# Autodesk Inventor assembly: Toughbox-mini box
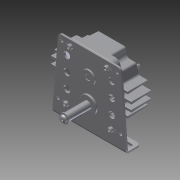
[picture p0: Inventor's stored thumbnail of the model, 180x180]
Saved by Autodesk Inventor 2014 SP1 (Build 180222100, 222)
## iProperties
Created: 2014-01-21
Part Number: Toughbox-mini box
Document SubType Name: Assembly
Designer: Nick
Translation Standard: STEP AP203
FileName: S:/Products/Gearboxes Spur Single Stage/Toughbox/Toughbox Mini/Toughbox-Mini.stp
PreProcessor: Unknown
PostProcessor: Build: 160, Release: 2012 RTM - Date: Tue 03/01/2011
Sent Units: millimeter
Uncertainty: 0.001
Author: Nick
## Documents named in this file (20)
- D:\Dropbox\School\PurdueFIRST\PFP Robot\PFP Robot with Cart\Toughbox-mini box.iam
- D:\Dropbox\School\PurdueFIRST\PFP Robot\PFP Robot with Cart\r6zz.ipt
- D:\Dropbox\School\PurdueFIRST\PFP Robot\PFP Robot with Cart\Toughbox_d03.ipt
- D:\Dropbox\School\PurdueFIRST\PFP Robot\PFP Robot with Cart\Toughbox_d07.ipt
- D:\Dropbox\School\PurdueFIRST\PFP Robot\PFP Robot with Cart\Toughbox_d05.ipt
- D:\Dropbox\School\PurdueFIRST\PFP Robot\PFP Robot with Cart\Toughbox_d08.ipt
- D:\Dropbox\School\PurdueFIRST\PFP Robot\PFP Robot with Cart\Toughbox_d06.ipt
- D:\Dropbox\School\PurdueFIRST\PFP Robot\PFP Robot with Cart\fr-6-zz.ipt
- D:\Dropbox\School\PurdueFIRST\PFP Robot\PFP Robot with Cart\fr-8-zz.ipt
- D:\Dropbox\School\PurdueFIRST\PFP Robot\PFP Robot with Cart\10-32_nylock_nut.ipt
- D:\Dropbox\School\PurdueFIRST\PFP Robot\PFP Robot with Cart\5-16_washer.ipt
- D:\Dropbox\School\PurdueFIRST\PFP Robot\PFP Robot with Cart\Toughbox_d09.ipt
- D:\Dropbox\School\PurdueFIRST\PFP Robot\PFP Robot with Cart\8mm_spring_clip.ipt
- D:\Dropbox\School\PurdueFIRST\PFP Robot\PFP Robot with Cart\Toughbox-mini_d01-5-12.ipt
- D:\Dropbox\School\PurdueFIRST\PFP Robot\PFP Robot with Cart\Toughbox-mini_d02.ipt
- D:\Dropbox\School\PurdueFIRST\PFP Robot\PFP Robot with Cart\250_washer.ipt
- D:\Dropbox\School\PurdueFIRST\PFP Robot\PFP Robot with Cart\14-20x0500_bhcs.ipt
- D:\Dropbox\School\PurdueFIRST\PFP Robot\PFP Robot with Cart\125x124x700_key.ipt
- D:\Dropbox\School\PurdueFIRST\PFP Robot\PFP Robot with Cart\10-32x0625_shcs.ipt
- D:\Dropbox\School\PurdueFIRST\PFP Robot\PFP Robot with Cart\TB Output Shaft AM14U.ipt
## Components (35 placed, 19 different names)
1. r6zz:1
2. r6zz:2
3. Toughbox_d03:1
4. Toughbox_d07:1
5. Toughbox_d05:1
6. Toughbox_d08:1
7. Toughbox_d06:1
8. fr-6-zz:1
9. fr-8-zz:1
10. 10-32_nylock_nut:1
11. 10-32_nylock_nut:2
12. 10-32_nylock_nut:3
13. 10-32_nylock_nut:4
14. 5-16_washer:1
15. 5-16_washer:2
16. 5-16_washer:3
17. 5-16_washer:4
18. Toughbox_d09:1
19. Toughbox_d09:2
20. 8mm_spring_clip:1
21. 8mm_spring_clip:2
22. Toughbox-mini_d01-5-12:1 — Insert:1
23. Toughbox-mini_d02:1
24. 250_washer:1
25. 14-20x0500_bhcs:1
26. 125x124x700_key:1
27. 10-32x0625_shcs:1
28. 10-32x0625_shcs:2
29. 10-32x0625_shcs:3
30. 10-32x0625_shcs:4
31. 10-32x0625_shcs:5
32. 10-32x0625_shcs:6
33. 10-32x0625_shcs:7
34. 10-32x0625_shcs:8
35. TB Output Shaft AM14U:1 — Insert:1
## Relationships (1: Insert 1)
- Insert:1 (-8.636 mm): Toughbox-mini_d01-5-12:1 ↔ TB Output Shaft AM14U:1
